# Autodesk Inventor assembly: Assembly20
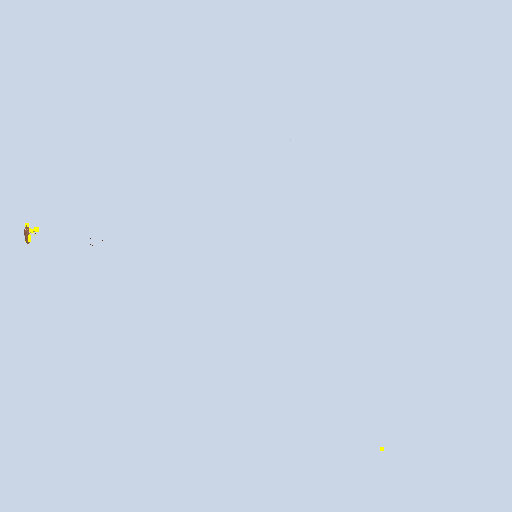
[picture p0: Inventor's stored thumbnail of the model, 512x512]
Saved by Autodesk Inventor 2024.1 (Build 281209000, 209)
## iProperties
Created: 2023-11-10
Part Number: Assembly20
Document SubType Name: Assembly
Designer: luvag
Author: luvag
## Documents named in this file (3)
- C:\Users\luvag\Desktop\Assembly20.iam
- C:\Users\luvag\Desktop\Assembly18.iam
- C:\Users\luvag\Desktop\trianglef.ipt
## Components (2 placed, 2 different names)
1. Assembly18:1 [sub-assembly]
2. trianglef:1
## Relationships (1: Mate 1)
- [Mate]: Assembly18:1 ↔ trianglef:1
